# Autodesk Inventor assembly: MG-Dribbler Zwischenzahnrad v2
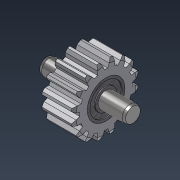
[picture p0: Inventor's stored thumbnail of the model, 180x180]
Saved by Autodesk Inventor 2022.2 (Build 262287010, 287A)
## iProperties
Part Number: MG-Dribbler Zwischenzahnrad v2
Material: Generisch
Document SubType Name: Assembly
Designer: rYan
Mass: 2.03629 g
Surface Area: 13.3279 cm^2
Volume: 0.647491 cm^3
Density: 3.1449 g/cm^3
Author: rYan
## Documents named in this file (4)
- D:\TIGERsGIT\Hardware\mechanik\2020\Inventor\Robot\Dribbler\MG-Dribbler Zwischenzahnrad v2.iam
- D:\TIGERsGIT\Hardware\mechanik\2020\Inventor\Purchased Parts\Zahnrad Polyketon z16 Modul 0.7.ipt
- D:\TIGERsGIT\Hardware\mechanik\2020\Inventor\Inhaltscenter\de-DE\ISO 2338(1)\DIN EN ISO 2338 - 3 m6 x 16.ipt
- D:\TIGERsGIT\Hardware\mechanik\2020\Inventor\Purchased Parts\Kugellager 683-ZZ.ipt
## Components (4 placed, 3 different names)
1. DIN EN ISO 2338 3 m6 x 16:1 — Einfügen:3, Fluchtend:1, Fluchtend:2, Fluchtend:3
2. Kugellager 683-ZZ:1 — Einfügen:4
3. Kugellager 683-ZZ:2 — Einfügen:3, Einfügen:4, Einfügen:5
4. Zahnrad Polyketon z16 Modul 0.7:1 — Einfügen:5
## Relationships (6: Insert 3, Flush 3)
- Einfügen:3 [Insert] (-5 mm): DIN EN ISO 2338 3 m6 x 16:1 ↔ Kugellager 683-ZZ:2
- Fluchtend:1 [Flush]: DIN EN ISO 2338 3 m6 x 16:1
- Fluchtend:2 [Flush]: DIN EN ISO 2338 3 m6 x 16:1
- Fluchtend:3 [Flush]: DIN EN ISO 2338 3 m6 x 16:1
- Einfügen:4 [Insert]: Kugellager 683-ZZ:1 ↔ Kugellager 683-ZZ:2
- Einfügen:5 [Insert]: Kugellager 683-ZZ:2 ↔ Zahnrad Polyketon z16 Modul 0.7:1
